# Autodesk Inventor assembly: Conic_Cover
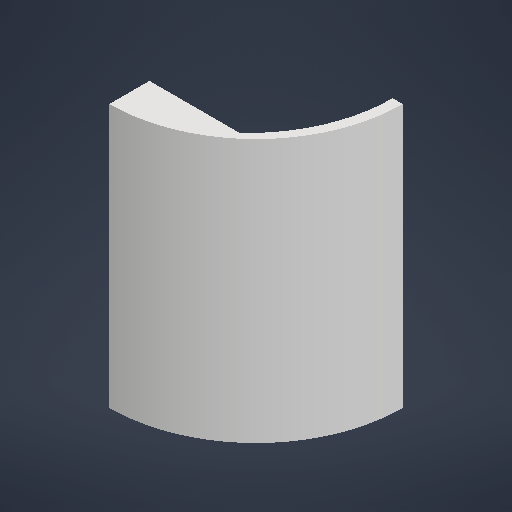
[picture p0: Inventor's stored thumbnail of the model, 512x512]
Saved by Autodesk Inventor 2026.2 (Build 302298000, 298)
## iProperties
Created: 2025-12-11
Part Number: Conic_Cover
Document SubType Name: Assembly
Designer: Thoma
Author: Thoma
## Documents named in this file (2)
- C:\Users\Thoma\OneDrive\Desktop\Inventor\Quarter_Open\Version_2\Conic_Cover.iam
- C:\Users\Thoma\OneDrive\Desktop\Inventor\Quarter_Open\Version_2\Conic_Cover_MIR.ipt
## Components (2 placed, 1 different names)
1. Conic_Cover_MIR:1 — Mate:1, Mate:2, Angle:1
2. Conic_Cover_MIR:2 — Mate:1, Mate:2, Angle:1
## Relationships (3: Mate 2, Angle 1)
- Mate:1: Conic_Cover_MIR:1 ↔ Conic_Cover_MIR:2
- Mate:2: Conic_Cover_MIR:1 ↔ Conic_Cover_MIR:2
- Angle:1 (0 deg): Conic_Cover_MIR:1 ↔ Conic_Cover_MIR:2
